# Autodesk Inventor assembly: J005356
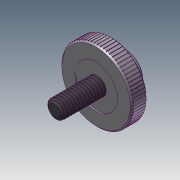
[picture p0: Inventor's stored thumbnail of the model, 180x180]
Saved by Autodesk Inventor 2015 SP1 (Build 190203100, 203)
## iProperties
Created: 2015-08-27
Vendor: HHMI: JRC - ID&F
Document SubType Name: Assembly
Designer: ARNOLDJ
Part Number: J005356
Description: THUMBSCREW ASSY HEADBAR CLAMP MBS POSITIONER
Project: P-201804
RuleStatus: InUse
AfterDocSave0: file://Part Number Cleaner
DESIGN DEPARTMENT: HHMI: JRC - ID&F
LAB/DEPT: SVOBODA (LAB)
REQUESTING SCIENTIST: SOFRONIEW, NICK
SPECIAL FINISH: NONE
SURFACE ROUGHNESS: N/A
ALTERED ITEM PART NUMBER: N/A
ALTERED ITEM VENDOR: N/A
ALTERED ITEM DESCRIPTION: N/A
Revision Number: -
## Documents named in this file (3)
- C:\_WORKSPACE\DATA\COLLABORATION\SVOBODA LAB\MOUSE POSITIONING SYSTEMS\MCAD\BALL SETUP\MBS POS-T-SCREW.iam
- C:\_WORKSPACE\DATA\COLLABORATION\SVOBODA LAB\MOUSE POSITIONING SYSTEMS\MCAD\BALL SETUP\MBS POS-T-SCREW BASE.ipt
- C:\_WORKSPACE\DATA\COLLABORATION\SVOBODA LAB\MOUSE POSITIONING SYSTEMS\MCAD\BALL SETUP\MBS 92290A148_AI.ipt
## Components (2 placed, 2 different names)
1. MBS POS-T-SCREW BASE:1 — Mate:2, Flush:1
2. MBS 92290A148_AI:1 — Mate:2, Flush:1
## Relationships (2: Mate 1, Flush 1)
- Mate:2: MBS POS-T-SCREW BASE:1 ↔ MBS 92290A148_AI:1
- Flush:1: MBS POS-T-SCREW BASE:1 ↔ MBS 92290A148_AI:1
